# Autodesk Inventor assembly: Assembly9 (Crank Case Sub Assembly)
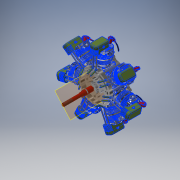
[picture p0: Inventor's stored thumbnail of the model, 180x180]
Saved by Autodesk Inventor 2018 (Build 220112000, 112)
## iProperties
Created: 2023-05-02
Part Number: Assembly9 (Crank Case Sub Assembly)
Document SubType Name: Assembly
Designer: Habib Mohamed
Author: Habib Mohamed
## Documents named in this file (5)
- D:\Inventor\My projects\Rotary Engine\Assembly\Assembly9 (Crank Case Sub Assembly).iam
- D:\Inventor\My projects\Rotary Engine\Main Block (Crank Case).ipt
- D:\Inventor\My projects\Rotary Engine\Assembly\Assembly8 (Cylinder Complete Sub Assembly).iam
- D:\Inventor\My projects\Rotary Engine\Assembly\Assembly6(Piston Sub Assembly Major).iam
- C:\Users\Habib Mohamed\Documents\Inventor\Content Center Files\R2018\en-US\ISO 4762(1)\DIN EN ISO 4762 - M4 x 12.ipt
## Components (37 placed, 4 different names)
1. Main Block (Crank Case):1 — Mate:1, Mate:2, Mate:3, Mate:4, Mate:6, Mate:7, Mate:8, Mate:9, Mate:10, Mate:11, Mate:12, Mate:13, Mate:14, Mate:16, Mate:18, Mate:20, Mate:22
2. Assembly6(Piston Sub Assembly Major):1 [sub-assembly] — Mate:1, Mate:5, Mate:6, Mate:7, Mate:8, Mate:9, Mate:10, Mate:11, Mate:12
3. Assembly8 (Cylinder Complete Sub Assembly):1 [sub-assembly] — Mate:2, Mate:3, Mate:4, Mate:5, Mate:13, Mate:15, Mate:17, Mate:19, Mate:21
4. DIN EN ISO 4762 M4 x 12:1 — Mate:14, Mate:15
5. DIN EN ISO 4762 M4 x 12:2 — Mate:16, Mate:17
6. DIN EN ISO 4762 M4 x 12:3 — Mate:18, Mate:19
7. DIN EN ISO 4762 M4 x 12:4 — Mate:20, Mate:21
8. Assembly8 (Cylinder Complete Sub Assembly):2 [sub-assembly]
9. DIN EN ISO 4762 M4 x 12:5
10. DIN EN ISO 4762 M4 x 12:6
11. DIN EN ISO 4762 M4 x 12:7
12. DIN EN ISO 4762 M4 x 12:8
13. Assembly8 (Cylinder Complete Sub Assembly):3 [sub-assembly]
14. DIN EN ISO 4762 M4 x 12:9
15. DIN EN ISO 4762 M4 x 12:10
16. DIN EN ISO 4762 M4 x 12:11
17. DIN EN ISO 4762 M4 x 12:12
18. Assembly8 (Cylinder Complete Sub Assembly):4 [sub-assembly]
19. DIN EN ISO 4762 M4 x 12:13
20. DIN EN ISO 4762 M4 x 12:14
21. DIN EN ISO 4762 M4 x 12:15
22. DIN EN ISO 4762 M4 x 12:16
23. Assembly8 (Cylinder Complete Sub Assembly):5 [sub-assembly]
24. DIN EN ISO 4762 M4 x 12:17
25. DIN EN ISO 4762 M4 x 12:18
26. DIN EN ISO 4762 M4 x 12:19
27. DIN EN ISO 4762 M4 x 12:20
28. Assembly8 (Cylinder Complete Sub Assembly):6 [sub-assembly]
29. DIN EN ISO 4762 M4 x 12:21
30. DIN EN ISO 4762 M4 x 12:22
31. DIN EN ISO 4762 M4 x 12:23
32. DIN EN ISO 4762 M4 x 12:24
33. Assembly8 (Cylinder Complete Sub Assembly):7 [sub-assembly]
34. DIN EN ISO 4762 M4 x 12:25
35. DIN EN ISO 4762 M4 x 12:26
36. DIN EN ISO 4762 M4 x 12:27
37. DIN EN ISO 4762 M4 x 12:28
## Component patterns: (7 elements, first: Assembly8 (Cylinder Complete Sub Assembly):1 + DIN EN ISO 4762 M4 x 12:1 + DIN EN ISO 4762 M4 x 12:2 + DIN EN ISO 4762 M4 x 12:3 + DIN EN ISO 4762 M4 x 12:4)
## Relationships (22: Mate 22)
- Mate:1: Main Block (Crank Case):1 ↔ Assembly6(Piston Sub Assembly Major):1
- Mate:2: Main Block (Crank Case):1 ↔ Assembly8 (Cylinder Complete Sub Assembly):1
- Mate:3: Main Block (Crank Case):1 ↔ Assembly8 (Cylinder Complete Sub Assembly):1
- Mate:4: Main Block (Crank Case):1 ↔ Assembly8 (Cylinder Complete Sub Assembly):1
- Mate:5: Assembly6(Piston Sub Assembly Major):1 ↔ Assembly8 (Cylinder Complete Sub Assembly):1
- Mate:6: Main Block (Crank Case):1 ↔ Assembly6(Piston Sub Assembly Major):1
- Mate:7: Main Block (Crank Case):1 ↔ Assembly6(Piston Sub Assembly Major):1
- Mate:8: Main Block (Crank Case):1 ↔ Assembly6(Piston Sub Assembly Major):1
- Mate:9: Main Block (Crank Case):1 ↔ Assembly6(Piston Sub Assembly Major):1
- Mate:10: Main Block (Crank Case):1 ↔ Assembly6(Piston Sub Assembly Major):1
- Mate:11: Main Block (Crank Case):1 ↔ Assembly6(Piston Sub Assembly Major):1
- Mate:12: Main Block (Crank Case):1 ↔ Assembly6(Piston Sub Assembly Major):1
- Mate:13: Main Block (Crank Case):1 ↔ Assembly8 (Cylinder Complete Sub Assembly):1
- Mate:14: Main Block (Crank Case):1 ↔ DIN EN ISO 4762 M4 x 12:1
- Mate:15: Assembly8 (Cylinder Complete Sub Assembly):1 ↔ DIN EN ISO 4762 M4 x 12:1
- Mate:16: Main Block (Crank Case):1 ↔ DIN EN ISO 4762 M4 x 12:2
- Mate:17: Assembly8 (Cylinder Complete Sub Assembly):1 ↔ DIN EN ISO 4762 M4 x 12:2
- Mate:18: Main Block (Crank Case):1 ↔ DIN EN ISO 4762 M4 x 12:3
- Mate:19: Assembly8 (Cylinder Complete Sub Assembly):1 ↔ DIN EN ISO 4762 M4 x 12:3
- Mate:20: Main Block (Crank Case):1 ↔ DIN EN ISO 4762 M4 x 12:4
- Mate:21: Assembly8 (Cylinder Complete Sub Assembly):1 ↔ DIN EN ISO 4762 M4 x 12:4
- Mate:22: Main Block (Crank Case):1
